# Autodesk Inventor assembly: Редуктор для двигателя
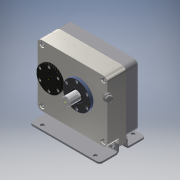
[picture p0: Inventor's stored thumbnail of the model, 180x180]
Saved by Autodesk Inventor 2016 (Build 200138000, 138)
## iProperties
Created: 2021-04-28
Part Number: Редуктор для двигателя
Material: Типовые
Document SubType Name: Assembly
Designer: Лол
Author: Лол
## Documents named in this file (34)
- C:\Users\Лол\Documents\Inventor\course_work\Редуктор для двигателя.iam
- C:\Users\Лол\Documents\Inventor\course_work\Корпус часть без резьбы.ipt
- C:\Users\Лол\Documents\Inventor\course_work\Подшипник\Подшипник-01.ipt
- C:\Users\Лол\Documents\Inventor\course_work\Подшипник.ipt
- C:\Users\Лол\Documents\Inventor\course_work\Подшипник\Подшипник-02.ipt
- C:\Users\Лол\Documents\Inventor\course_work\Быстроходный вал.ipt
- C:\Users\Лол\Documents\Inventor\course_work\Тихоходный вал.ipt
- C:\Users\Лол\Documents\Inventor\course_work\Кольцо A30 ГОСТ 13942-86.ipt
- C:\Users\Лол\Documents\Inventor\course_work\Кольцо A35 ГОСТ 13942-86.ipt
- C:\Users\Лол\Documents\Inventor\course_work\Тихоходное колесо.ipt
- C:\Users\Лол\Documents\Inventor\course_work\Корпус центральная часть.ipt
- C:\Users\Лол\Documents\Inventor\course_work\Корпус часть с резьбой.ipt
- C:\Users\Лол\Documents\Inventor\course_work\Гайка M30x1.5 6H ГОСТ 6393-73.ipt
- C:\Users\Лол\Documents\Inventor\course_work\Гайка M33x1.5 6H ГОСТ 6393-73.ipt
- C:\Users\Лол\Documents\Inventor\course_work\ISO 2340 - A - 6 x 40ISO.ipt
- C:\Users\Лол\Documents\Inventor\course_work\AS 1420 - 1973 - M10 x 75.ipt
- C:\Users\Лол\Documents\Inventor\course_work\Крышка маленькая_62.ipt
- C:\Users\Лол\Documents\Inventor\course_work\КОЛЬЦО 062-066-25 гост 9833.ipt
- C:\Users\Лол\Documents\Inventor\course_work\Манжет 1-30x72x10 ГОСТ 8752-79.ipt
- C:\Users\Лол\Documents\Inventor\course_work\Манжет 1-28x62x10 ГОСТ 8752-79.ipt
- C:\Users\Лол\Documents\Inventor\course_work\Крышка большая_72.ipt
- C:\Users\Лол\Documents\Inventor\course_work\КОЛЬЦО 072-066-25 гост 9833.ipt
- C:\Users\Лол\Documents\Inventor\course_work\AS 1420 - 1973 - M6 x 12.ipt
- C:\Users\Лол\Documents\Inventor\course_work\Крышка маленькая_под манж_01.ipt
- C:\Users\Лол\Documents\Inventor\course_work\Крышка большая_ПОД МАНЖЕТУ.ipt
- C:\Users\Лол\Documents\Inventor\course_work\Манжет 1-28x40x7 ГОСТ 8752-79.ipt
- C:\Users\Лол\Documents\Inventor\course_work\Манжет 1-30x42x7 ГОСТ 8752-79.ipt
- C:\Users\Лол\Documents\Inventor\course_work\ОПОРА_05.ipt
- C:\Users\Лол\Documents\Inventor\Content Center Files\R2016\ru-RU\Bolt GOST R 50274-92\Болт M10-6g×50-F ГОСТ Р 50274-92.ipt
- C:\Users\Лол\Documents\Inventor\Content Center Files\R2016\ru-RU\Washer 1 GOST 6402-78\Шайба 10Л ГОСТ 6402-78.ipt
- C:\Users\Лол\Documents\Inventor\Content Center Files\R2016\ru-RU\GOST 2524-70\Гайка M10-6H ГОСТ 2524-70.ipt
- C:\Users\Лол\Documents\Inventor\Content Center Files\R2016\ru-RU\GOST 23360-78 (1)\Шпонка 8x7x28 ГОСТ 23360-78.ipt
- C:\Users\Лол\Documents\Inventor\Content Center Files\R2016\ru-RU\CSN 02 1915.21  FT\CSN 02 1915.21 - M 20 x 10.ipt
- C:\Users\Лол\Documents\Inventor\Content Center Files\R2016\ru-RU\DIN 7603 A\DIN 7603 - A22 x 27  (lt).ipt
## Components (78 placed, 32 different names)
1. Корпус часть без резьбы:1 — Заподлицо:1, Заподлицо:2, Заподлицо:3, Совмещение:1, Совмещение:2, Совмещение:3, Совмещение:4, Совмещение:14, Совмещение:27, Совмещение:28, Совмещение:33, Совмещение:34, Совмещение:35, Совмещение:36, Совмещение:37, Совмещение:38, Совмещение:39, Совмещение:40, Совмещение:43, Совмещение:44, Совмещение:46, Заподлицо:4, Совмещение:61, Совмещение:62, Совмещение:82, Совмещение:83, Совмещение:84
2. Подшипник-01:1 — Совмещение:18, Совмещение:19, Совмещение:22, Совмещение:24
3. Подшипник-01:2 — Совмещение:1, Совмещение:2, Совмещение:5, Совмещение:13
4. Подшипник-02:3 — Совмещение:3, Совмещение:4, Совмещение:6, Совмещение:26
5. Подшипник-02:4 — Совмещение:16, Совмещение:17, Совмещение:, Совмещение:88
6. Быстроходный вал:1 — Совмещение:5, Совмещение:7, Совмещение:8, Совмещение:22, Совмещение:23, Совмещение:85, Угол:1, Совмещение:157, Совмещение:158
7. Тихоходный вал:1 — Совмещение:6, Совмещение:9, Совмещение:12, Совмещение:25, Совмещение:48, Совмещение:87, Совмещение:88, Совмещение:112, Совмещение:149, Совмещение:150, Совмещение:151
8. Кольцо A30 ГОСТ 13942-86:1 — Совмещение:7, Совмещение:8, Совмещение:13
9. Кольцо A35 ГОСТ 13942-86:1 — Совмещение:9, Совмещение:, Совмещение:48
10. Тихоходное колесо:2 — Совмещение:12, Совмещение:87
11. Корпус центральная часть:1 — Совмещение:14, Совмещение:15, Совмещение:29, Совмещение:30, Совмещение:31, Совмещение:32, Совмещение:91, Заподлицо:8, Совмещение:92, Совмещение:93, Совмещение:94, Совмещение:95, Совмещение:96, Заподлицо:9, Совмещение:114, Совмещение:115, Совмещение:116, Совмещение:117, Совмещение:118, Совмещение:119, Совмещение:124, Совмещение:125
12. Корпус часть с резьбой:1 — Совмещение:15, Совмещение:16, Совмещение:17, Совмещение:18, Совмещение:19, Совмещение:47, Заподлицо:5, Совмещение:49, Совмещение:56, Совмещение:57, Совмещение:65, Совмещение:79, Совмещение:80, Совмещение:81, Угол:1
13. Гайка M30x1.5 6H ГОСТ 6393-73:1 — Совмещение:23, Совмещение:24
14. Гайка M33x1.5 6H ГОСТ 6393-73:1 — Совмещение:25, Совмещение:26
15. ISO 2340 - A - 6 x 40ISO:1 — Совмещение:27, Совмещение:29, Совмещение:31
16. ISO 2340 - A - 6 x 40ISO:2 — Совмещение:28, Совмещение:30, Совмещение:32
17. AS 1420 - 1973 - M10 x 75:1 — Совмещение:33, Совмещение:34
18. AS 1420 - 1973 - M10 x 75:2 — Совмещение:35, Совмещение:36
19. AS 1420 - 1973 - M10 x 75:3 — Совмещение:37, Совмещение:38
20. AS 1420 - 1973 - M10 x 75:4 — Совмещение:39, Совмещение:40
21. Крышка маленькая_62:1 — Совмещение:41, Совмещение:42, Совмещение:43, Совмещение:44, Совмещение:61, Совмещение:63, Совмещение:64
22. КОЛЬЦО 062-066-25 гост 9833:1 — Совмещение:41, Совмещение:42
23. Манжет 1-30x72x10 ГОСТ 8752-79:2 — Совмещение:46, Заподлицо:4
24. Манжет 1-28x62x10 ГОСТ 8752-79:2 — Совмещение:47, Заподлицо:5
25. Крышка большая_72:2 — Совмещение:49, Совмещение:50, Совмещение:51, Совмещение:56, Совмещение:57, Совмещение:60, Совмещение:66
26. КОЛЬЦО 072-066-25 гост 9833:1 — Совмещение:50, Совмещение:51
27. Крышка маленькая_под манж_01:1 — Совмещение:79, Совмещение:80, Совмещение:81, Заподлицо:6, Совмещение:105, Совмещение:106, Совмещение:107, Совмещение:108
28. Крышка большая_ПОД МАНЖЕТУ:1 — Совмещение:82, Совмещение:83, Совмещение:84, Заподлицо:7, Совмещение:86, Совмещение:103, Совмещение:104, Совмещение:110, Совмещение:111
29. Манжет 1-28x40x7 ГОСТ 8752-79:2 — Совмещение:85, Заподлицо:6
30. Манжет 1-30x42x7 ГОСТ 8752-79:1 — Заподлицо:7, Совмещение:86
31. ISO 2340 - A - 6 x 40ISO:3 — Совмещение:91, Заподлицо:8
32. ISO 2340 - A - 6 x 40ISO:4 — Совмещение:92, Совмещение:95
33. ISO 2340 - A - 6 x 40ISO:5 — Совмещение:93, Совмещение:96
34. ISO 2340 - A - 6 x 40ISO:6 — Совмещение:94, Заподлицо:9
35. КОЛЬЦО 072-066-25 гост 9833:2 — Совмещение:103, Совмещение:104
36. КОЛЬЦО 062-066-25 гост 9833:2 — Совмещение:105, Совмещение:106
37. ОПОРА_05:1 — Совмещение:114, Совмещение:115, Совмещение:116, Совмещение:120, Совмещение:121, Совмещение:122, Совмещение:123, Совмещение:126, Совмещение:127
38. ОПОРА_05:2 — Совмещение:117, Совмещение:118, Совмещение:119, Совмещение:132, Совмещение:133, Совмещение:134, Совмещение:135
39. Болт ГОСТ Р 50274-92 M10-6g×50-F:1 — Совмещение:120, Совмещение:121, Совмещение:128, Совмещение:136
40. Болт ГОСТ Р 50274-92 M10-6g×50-F:2 — Совмещение:125, Совмещение:127, Совмещение:131, Совмещение:139
41. Болт ГОСТ Р 50274-92 M10-6g×50-F:3 — Совмещение:124, Совмещение:126, Совмещение:130, Совмещение:138
42. Болт ГОСТ Р 50274-92 M10-6g×50-F:4 — Совмещение:122, Совмещение:123, Совмещение:129, Совмещение:137
43. Шайба 1 ГОСТ 6402-78 10Л:1 — Совмещение:128, Совмещение:132, Совмещение:140
44. Шайба 1 ГОСТ 6402-78 10Л:2 — Совмещение:129, Совмещение:133, Совмещение:141
45. Шайба 1 ГОСТ 6402-78 10Л:3 — Совмещение:130, Совмещение:135, Совмещение:142
46. Шайба 1 ГОСТ 6402-78 10Л:4 — Совмещение:131, Совмещение:134, Совмещение:143
47. Гайка ГОСТ 2524-70 M10:1 — Совмещение:136, Совмещение:140
48. Гайка ГОСТ 2524-70 M10:2 — Совмещение:137, Совмещение:141
49. Гайка ГОСТ 2524-70 M10:3 — Совмещение:138, Совмещение:142
50. Гайка ГОСТ 2524-70 M10:4 — Совмещение:139, Совмещение:143
51. Шпонка ГОСТ 23360-78 8 x 7 x 28:1 — Совмещение:149, Совмещение:150, Совмещение:151
52. Шпонка ГОСТ 23360-78 8 x 7 x 28:2 — Совмещение:157, Совмещение:158
53. CSN 02 1915.21 (мелкая резьба) M 20 x 10:1 — Совмещение:155, Совмещение:156
54. DIN 7603 A A22 x 27  (lt):1 — Совмещение:155, Совмещение:156
55. AS 1420 - 1973 - M6 x 12:1 — Совмещение:62, Совмещение:63
56. AS 1420 - 1973 - M6 x 12:2
57. AS 1420 - 1973 - M6 x 12:3
58. AS 1420 - 1973 - M6 x 12:4
59. AS 1420 - 1973 - M6 x 12:5
60. AS 1420 - 1973 - M6 x 12:6
61. AS 1420 - 1973 - M6 x 12:8 — Совмещение:65, Совмещение:66
62. AS 1420 - 1973 - M6 x 12:9
63. AS 1420 - 1973 - M6 x 12:10
64. AS 1420 - 1973 - M6 x 12:11
65. AS 1420 - 1973 - M6 x 12:12
66. AS 1420 - 1973 - M6 x 12:13
67. AS 1420 - 1973 - M6 x 12:15 — Совмещение:107, Совмещение:108
68. AS 1420 - 1973 - M6 x 12:16
69. AS 1420 - 1973 - M6 x 12:17
70. AS 1420 - 1973 - M6 x 12:18
71. AS 1420 - 1973 - M6 x 12:19
72. AS 1420 - 1973 - M6 x 12:20
73. AS 1420 - 1973 - M6 x 12:14 — Совмещение:110, Совмещение:111
74. AS 1420 - 1973 - M6 x 12:21
75. AS 1420 - 1973 - M6 x 12:22
76. AS 1420 - 1973 - M6 x 12:23
77. AS 1420 - 1973 - M6 x 12:24
78. AS 1420 - 1973 - M6 x 12:25
## Component patterns: (6 elements, first: AS 1420 - 1973 - M6 x 12:1), (6 elements, first: AS 1420 - 1973 - M6 x 12:8), (6 elements, first: AS 1420 - 1973 - M6 x 12:15), (6 elements, first: AS 1420 - 1973 - M6 x 12:14)
## Relationships (128: Mate 118, Flush 9, Angle 1)
- Заподлицо:1 [Flush]: Корпус часть без резьбы:1
- Заподлицо:2 [Flush] (-37.142 mm): Корпус часть без резьбы:1
- Заподлицо:3 [Flush] (-27.571 mm): Корпус часть без резьбы:1
- Совмещение:1 [Mate]: Корпус часть без резьбы:1 ↔ Подшипник-01:2
- Совмещение:2 [Mate]: Корпус часть без резьбы:1 ↔ Подшипник-01:2
- Совмещение:3 [Mate]: Корпус часть без резьбы:1 ↔ Подшипник-02:3
- Совмещение:4 [Mate]: Корпус часть без резьбы:1 ↔ Подшипник-02:3
- Совмещение:5 [Mate]: Подшипник-01:2 ↔ Быстроходный вал:1
- Совмещение:6 [Mate]: Подшипник-02:3 ↔ Тихоходный вал:1
- Совмещение:7 [Mate]: Быстроходный вал:1 ↔ Кольцо A30 ГОСТ 13942-86:1
- Совмещение:8 [Mate]: Быстроходный вал:1 ↔ Кольцо A30 ГОСТ 13942-86:1
- Совмещение:9 [Mate]: Тихоходный вал:1 ↔ Кольцо A35 ГОСТ 13942-86:1
- Совмещение:12 [Mate]: Тихоходный вал:1 ↔ Тихоходное колесо:2
- Совмещение:13 [Mate]: Подшипник-01:2 ↔ Кольцо A30 ГОСТ 13942-86:1
- Совмещение:14 [Mate]: Корпус часть без резьбы:1 ↔ Корпус центральная часть:1
- Совмещение:15 [Mate]: Корпус центральная часть:1 ↔ Корпус часть с резьбой:1
- Совмещение:16 [Mate]: Подшипник-02:4 ↔ Корпус часть с резьбой:1
- Совмещение:17 [Mate]: Подшипник-02:4 ↔ Корпус часть с резьбой:1
- Совмещение:18 [Mate]: Подшипник-01:1 ↔ Корпус часть с резьбой:1
- Совмещение:19 [Mate]: Подшипник-01:1 ↔ Корпус часть с резьбой:1
- Совмещение: [Mate]: Подшипник-02:4 ↔ Кольцо A35 ГОСТ 13942-86:1
- Совмещение:22 [Mate]: Подшипник-01:1 ↔ Быстроходный вал:1
- Совмещение:23 [Mate]: Быстроходный вал:1 ↔ Гайка M30x1.5 6H ГОСТ 6393-73:1
- Совмещение:24 [Mate]: Подшипник-01:1 ↔ Гайка M30x1.5 6H ГОСТ 6393-73:1
- Совмещение:25 [Mate]: Тихоходный вал:1 ↔ Гайка M33x1.5 6H ГОСТ 6393-73:1
- Совмещение:26 [Mate]: Подшипник-02:3 ↔ Гайка M33x1.5 6H ГОСТ 6393-73:1
- Совмещение:27 [Mate]: Корпус часть без резьбы:1 ↔ ISO 2340 - A - 6 x 40ISO:1
- Совмещение:28 [Mate]: Корпус часть без резьбы:1 ↔ ISO 2340 - A - 6 x 40ISO:2
- Совмещение:29 [Mate]: Корпус центральная часть:1 ↔ ISO 2340 - A - 6 x 40ISO:1
- Совмещение:30 [Mate]: Корпус центральная часть:1 ↔ ISO 2340 - A - 6 x 40ISO:2
- Совмещение:31 [Mate] (7.5 mm): Корпус центральная часть:1 ↔ ISO 2340 - A - 6 x 40ISO:1
- Совмещение:32 [Mate] (7.5 mm): Корпус центральная часть:1 ↔ ISO 2340 - A - 6 x 40ISO:2
- Совмещение:33 [Mate]: Корпус часть без резьбы:1 ↔ AS 1420 - 1973 - M10 x 75:1
- Совмещение:34 [Mate]: Корпус часть без резьбы:1 ↔ AS 1420 - 1973 - M10 x 75:1
- Совмещение:35 [Mate]: Корпус часть без резьбы:1 ↔ AS 1420 - 1973 - M10 x 75:2
- Совмещение:36 [Mate]: Корпус часть без резьбы:1 ↔ AS 1420 - 1973 - M10 x 75:2
- Совмещение:37 [Mate]: Корпус часть без резьбы:1 ↔ AS 1420 - 1973 - M10 x 75:3
- Совмещение:38 [Mate]: Корпус часть без резьбы:1 ↔ AS 1420 - 1973 - M10 x 75:3
- Совмещение:39 [Mate]: Корпус часть без резьбы:1 ↔ AS 1420 - 1973 - M10 x 75:4
- Совмещение:40 [Mate]: Корпус часть без резьбы:1 ↔ AS 1420 - 1973 - M10 x 75:4
- Совмещение:41 [Mate]: Крышка маленькая_62:1 ↔ КОЛЬЦО 062-066-25 гост 9833:1
- Совмещение:42 [Mate] (1.25 mm): Крышка маленькая_62:1 ↔ КОЛЬЦО 062-066-25 гост 9833:1
- Совмещение:43 [Mate]: Корпус часть без резьбы:1 ↔ Крышка маленькая_62:1
- Совмещение:44 [Mate]: Корпус часть без резьбы:1 ↔ Крышка маленькая_62:1
- Совмещение:46 [Mate]: Корпус часть без резьбы:1 ↔ Манжет 1-30x72x10 ГОСТ 8752-79:2
- Заподлицо:4 [Flush]: Корпус часть без резьбы:1 ↔ Манжет 1-30x72x10 ГОСТ 8752-79:2
- Совмещение:47 [Mate]: Корпус часть с резьбой:1 ↔ Манжет 1-28x62x10 ГОСТ 8752-79:2
- Заподлицо:5 [Flush]: Корпус часть с резьбой:1 ↔ Манжет 1-28x62x10 ГОСТ 8752-79:2
- Совмещение:48 [Mate]: Тихоходный вал:1 ↔ Кольцо A35 ГОСТ 13942-86:1
- Совмещение:49 [Mate]: Корпус часть с резьбой:1 ↔ Крышка большая_72:2
- Совмещение:50 [Mate]: Крышка большая_72:2 ↔ КОЛЬЦО 072-066-25 гост 9833:1
- Совмещение:51 [Mate] (1.25 mm): Крышка большая_72:2 ↔ КОЛЬЦО 072-066-25 гост 9833:1
- Совмещение:56 [Mate]: Корпус часть с резьбой:1 ↔ Крышка большая_72:2
- Совмещение:57 [Mate]: Корпус часть с резьбой:1 ↔ Крышка большая_72:2
- Совмещение:60 [Mate]: Крышка большая_72:2
- Совмещение:61 [Mate]: Корпус часть без резьбы:1 ↔ Крышка маленькая_62:1
- Совмещение:62 [Mate]: Корпус часть без резьбы:1 ↔ AS 1420 - 1973 - M6 x 12:1
- Совмещение:63 [Mate]: Крышка маленькая_62:1 ↔ AS 1420 - 1973 - M6 x 12:1
- Совмещение:64 [Mate]: Крышка маленькая_62:1
- Совмещение:65 [Mate]: Корпус часть с резьбой:1 ↔ AS 1420 - 1973 - M6 x 12:8
- Совмещение:66 [Mate]: Крышка большая_72:2 ↔ AS 1420 - 1973 - M6 x 12:8
- Совмещение:79 [Mate]: Корпус часть с резьбой:1 ↔ Крышка маленькая_под манж_01:1
- Совмещение:80 [Mate]: Корпус часть с резьбой:1 ↔ Крышка маленькая_под манж_01:1
- Совмещение:81 [Mate]: Корпус часть с резьбой:1 ↔ Крышка маленькая_под манж_01:1
- Совмещение:82 [Mate]: Корпус часть без резьбы:1 ↔ Крышка большая_ПОД МАНЖЕТУ:1
- Совмещение:83 [Mate]: Корпус часть без резьбы:1 ↔ Крышка большая_ПОД МАНЖЕТУ:1
- Совмещение:84 [Mate]: Корпус часть без резьбы:1 ↔ Крышка большая_ПОД МАНЖЕТУ:1
- Совмещение:85 [Mate]: Быстроходный вал:1 ↔ Манжет 1-28x40x7 ГОСТ 8752-79:2
- Заподлицо:6 [Flush]: Крышка маленькая_под манж_01:1 ↔ Манжет 1-28x40x7 ГОСТ 8752-79:2
- Заподлицо:7 [Flush]: Крышка большая_ПОД МАНЖЕТУ:1 ↔ Манжет 1-30x42x7 ГОСТ 8752-79:1
- Совмещение:86 [Mate]: Крышка большая_ПОД МАНЖЕТУ:1 ↔ Манжет 1-30x42x7 ГОСТ 8752-79:1
- Совмещение:87 [Mate]: Тихоходный вал:1 ↔ Тихоходное колесо:2
- Совмещение:88 [Mate]: Подшипник-02:4 ↔ Тихоходный вал:1
- Совмещение:91 [Mate]: Корпус центральная часть:1 ↔ ISO 2340 - A - 6 x 40ISO:3
- Заподлицо:8 [Flush] (7.5 mm): Корпус центральная часть:1 ↔ ISO 2340 - A - 6 x 40ISO:3
- Совмещение:92 [Mate]: Корпус центральная часть:1 ↔ ISO 2340 - A - 6 x 40ISO:4
- Совмещение:93 [Mate]: Корпус центральная часть:1 ↔ ISO 2340 - A - 6 x 40ISO:5
- Совмещение:94 [Mate]: Корпус центральная часть:1 ↔ ISO 2340 - A - 6 x 40ISO:6
- Совмещение:95 [Mate] (7.5 mm): Корпус центральная часть:1 ↔ ISO 2340 - A - 6 x 40ISO:4
- Совмещение:96 [Mate] (7.5 mm): Корпус центральная часть:1 ↔ ISO 2340 - A - 6 x 40ISO:5
- Заподлицо:9 [Flush] (7.5 mm): Корпус центральная часть:1 ↔ ISO 2340 - A - 6 x 40ISO:6
- Совмещение:103 [Mate]: Крышка большая_ПОД МАНЖЕТУ:1 ↔ КОЛЬЦО 072-066-25 гост 9833:2
- Совмещение:104 [Mate] (1.25 mm): Крышка большая_ПОД МАНЖЕТУ:1 ↔ КОЛЬЦО 072-066-25 гост 9833:2
- Совмещение:105 [Mate]: Крышка маленькая_под манж_01:1 ↔ КОЛЬЦО 062-066-25 гост 9833:2
- Совмещение:106 [Mate] (1.25 mm): Крышка маленькая_под манж_01:1 ↔ КОЛЬЦО 062-066-25 гост 9833:2
- Совмещение:107 [Mate]: Крышка маленькая_под манж_01:1 ↔ AS 1420 - 1973 - M6 x 12:15
- Совмещение:108 [Mate]: Крышка маленькая_под манж_01:1 ↔ AS 1420 - 1973 - M6 x 12:15
- Совмещение:110 [Mate]: Крышка большая_ПОД МАНЖЕТУ:1 ↔ AS 1420 - 1973 - M6 x 12:14
- Совмещение:111 [Mate]: Крышка большая_ПОД МАНЖЕТУ:1 ↔ AS 1420 - 1973 - M6 x 12:14
- Совмещение:112 [Mate]: Тихоходный вал:1
- Совмещение:114 [Mate]: Корпус центральная часть:1 ↔ ОПОРА_05:1
- Совмещение:115 [Mate]: Корпус центральная часть:1 ↔ ОПОРА_05:1
- Совмещение:116 [Mate]: Корпус центральная часть:1 ↔ ОПОРА_05:1
- Совмещение:117 [Mate]: Корпус центральная часть:1 ↔ ОПОРА_05:2
- Совмещение:118 [Mate]: Корпус центральная часть:1 ↔ ОПОРА_05:2
- Совмещение:119 [Mate]: Корпус центральная часть:1 ↔ ОПОРА_05:2
- Совмещение:120 [Mate]: ОПОРА_05:1 ↔ Болт ГОСТ Р 50274-92 M10-6g×50-F:1
- Совмещение:121 [Mate]: ОПОРА_05:1 ↔ Болт ГОСТ Р 50274-92 M10-6g×50-F:1
- Совмещение:122 [Mate]: ОПОРА_05:1 ↔ Болт ГОСТ Р 50274-92 M10-6g×50-F:4
- Совмещение:123 [Mate]: ОПОРА_05:1 ↔ Болт ГОСТ Р 50274-92 M10-6g×50-F:4
- Совмещение:124 [Mate]: Корпус центральная часть:1 ↔ Болт ГОСТ Р 50274-92 M10-6g×50-F:3
- Совмещение:125 [Mate]: Корпус центральная часть:1 ↔ Болт ГОСТ Р 50274-92 M10-6g×50-F:2
- Совмещение:126 [Mate]: ОПОРА_05:1 ↔ Болт ГОСТ Р 50274-92 M10-6g×50-F:3
- Совмещение:127 [Mate]: ОПОРА_05:1 ↔ Болт ГОСТ Р 50274-92 M10-6g×50-F:2
- Совмещение:128 [Mate]: Болт ГОСТ Р 50274-92 M10-6g×50-F:1 ↔ Шайба 1 ГОСТ 6402-78 10Л:1
- Совмещение:129 [Mate]: Болт ГОСТ Р 50274-92 M10-6g×50-F:4 ↔ Шайба 1 ГОСТ 6402-78 10Л:2
- Совмещение:130 [Mate]: Болт ГОСТ Р 50274-92 M10-6g×50-F:3 ↔ Шайба 1 ГОСТ 6402-78 10Л:3
- Совмещение:131 [Mate]: Болт ГОСТ Р 50274-92 M10-6g×50-F:2 ↔ Шайба 1 ГОСТ 6402-78 10Л:4
- Совмещение:132 [Mate]: ОПОРА_05:2 ↔ Шайба 1 ГОСТ 6402-78 10Л:1
- Совмещение:133 [Mate]: ОПОРА_05:2 ↔ Шайба 1 ГОСТ 6402-78 10Л:2
- Совмещение:134 [Mate]: ОПОРА_05:2 ↔ Шайба 1 ГОСТ 6402-78 10Л:4
- Совмещение:135 [Mate]: ОПОРА_05:2 ↔ Шайба 1 ГОСТ 6402-78 10Л:3
- Совмещение:136 [Mate]: Болт ГОСТ Р 50274-92 M10-6g×50-F:1 ↔ Гайка ГОСТ 2524-70 M10:1
- Совмещение:137 [Mate]: Болт ГОСТ Р 50274-92 M10-6g×50-F:4 ↔ Гайка ГОСТ 2524-70 M10:2
- Совмещение:138 [Mate]: Болт ГОСТ Р 50274-92 M10-6g×50-F:3 ↔ Гайка ГОСТ 2524-70 M10:3
- Совмещение:139 [Mate]: Болт ГОСТ Р 50274-92 M10-6g×50-F:2 ↔ Гайка ГОСТ 2524-70 M10:4
- Совмещение:140 [Mate]: Шайба 1 ГОСТ 6402-78 10Л:1 ↔ Гайка ГОСТ 2524-70 M10:1
- Совмещение:141 [Mate]: Шайба 1 ГОСТ 6402-78 10Л:2 ↔ Гайка ГОСТ 2524-70 M10:2
- Совмещение:142 [Mate]: Шайба 1 ГОСТ 6402-78 10Л:3 ↔ Гайка ГОСТ 2524-70 M10:3
- Совмещение:143 [Mate]: Шайба 1 ГОСТ 6402-78 10Л:4 ↔ Гайка ГОСТ 2524-70 M10:4
- Совмещение:149 [Mate]: Тихоходный вал:1 ↔ Шпонка ГОСТ 23360-78 8 x 7 x 28:1
- Совмещение:150 [Mate]: Тихоходный вал:1 ↔ Шпонка ГОСТ 23360-78 8 x 7 x 28:1
- Совмещение:151 [Mate]: Тихоходный вал:1 ↔ Шпонка ГОСТ 23360-78 8 x 7 x 28:1
- Совмещение:155 [Mate]: CSN 02 1915.21 (мелкая резьба) M 20 x 10:1 ↔ DIN 7603 A A22 x 27  (lt):1
- Совмещение:156 [Mate]: CSN 02 1915.21 (мелкая резьба) M 20 x 10:1 ↔ DIN 7603 A A22 x 27  (lt):1
- Угол:1 [Angle] (120 deg): Быстроходный вал:1 ↔ Корпус часть с резьбой:1
- Совмещение:157 [Mate]: Быстроходный вал:1 ↔ Шпонка ГОСТ 23360-78 8 x 7 x 28:2
- Совмещение:158 [Mate]: Быстроходный вал:1 ↔ Шпонка ГОСТ 23360-78 8 x 7 x 28:2
